# Autodesk Inventor assembly: ModulWalkaNapinajacego
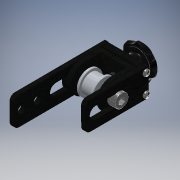
[picture p0: Inventor's stored thumbnail of the model, 180x180]
Saved by Autodesk Inventor 2019 (Build 230136000, 136)
## iProperties
Created: 2020-08-21
Part Number: ModulWalkaNapinajacego
Document SubType Name: Assembly
Designer: estee
Author: estee
## Documents named in this file (9)
- C:\Users\estee\OneDrive\Pulpit\estere\1\MUM\nowygit\Mechanika\Moduł obrotu RET Estera\projejt\projejt\ModulWalkaNapinajacego.iam
- C:\Users\estee\OneDrive\Pulpit\estere\1\MUM\nowygit\Mechanika\Moduł obrotu RET Estera\projejt\projejt\Ramka1.ipt
- C:\Users\estee\OneDrive\Pulpit\estere\1\MUM\nowygit\Mechanika\Moduł obrotu RET Estera\projejt\projejt\Ramka2.ipt
- C:\Users\estee\OneDrive\Pulpit\estere\1\MUM\nowygit\Mechanika\Moduł obrotu RET Estera\projejt\projejt\Ramka3.ipt
- C:\Users\estee\OneDrive\Pulpit\estere\1\MUM\nowygit\Mechanika\Moduł obrotu RET Estera\projejt\projejt\Ramka4.ipt
- C:\Users\estee\OneDrive\Dokumenty\Inventor\Content Center Files\R2019\en-US\BS EN ISO 7045 H\EN ISO 7045 - M2 x 6 - 4.8 - H(1).ipt
- C:\Users\estee\OneDrive\Pulpit\estere\1\MUM\nowygit\Mechanika\Moduł obrotu RET Estera\projejt\projejt\ModulKolaNapinajacego.iam
- C:\Users\estee\OneDrive\Dokumenty\Inventor\Star Knob M6 Male.ipt
- C:\Users\estee\OneDrive\Pulpit\estere\1\MUM\nowygit\Mechanika\Moduł obrotu RET Estera\projejt\projejt\WkretDoNapinacza.ipt
## Components (11 placed, 8 different names)
1. Ramka1:1 — Mate:1, Mate:2, Flush:1, Mate:3, Mate:4, Flush:2, Mate:6, Mate:19, Mate:20, Mate:21, Mate:22
2. Ramka2:1 — Mate:1, Mate:2, Flush:1, Mate:5, Mate:7, Mate:8, Mate:13, Mate:14
3. Ramka3:1 — Mate:3, Mate:4, Flush:2, Mate:9, Mate:10, Mate:11, Mate:12
4. Ramka4:1 — Mate:5, Mate:6, Mate:15, Mate:16
5. BS EN ISO 7045 H - Metric M2 x 6 - 4.8 - H:1 — Mate:7, Mate:13
6. BS EN ISO 7045 H - Metric M2 x 6 - 4.8 - H:2 — Mate:8, Mate:14
7. BS EN ISO 7045 H - Metric M2 x 6 - 4.8 - H:3 — Mate:9, Mate:11
8. BS EN ISO 7045 H - Metric M2 x 6 - 4.8 - H:4 — Mate:10, Mate:12
9. ModulKolaNapinajacego:1 [sub-assembly] — Mate:19, Mate:20
10. Star Knob M6 Male:1 — Mate:15, Mate:16
11. WkretDoNapinacza:1 — Mate:21, Mate:22
## Relationships (22: Mate 20, Flush 2)
- Mate:1: Ramka1:1 ↔ Ramka2:1
- Mate:2: Ramka1:1 ↔ Ramka2:1
- Flush:1: Ramka1:1 ↔ Ramka2:1
- Mate:3: Ramka1:1 ↔ Ramka3:1
- Mate:4: Ramka1:1 ↔ Ramka3:1
- Flush:2: Ramka1:1 ↔ Ramka3:1
- Mate:5: Ramka2:1 ↔ Ramka4:1
- Mate:6: Ramka1:1 ↔ Ramka4:1
- Mate:7: Ramka2:1 ↔ BS EN ISO 7045 H - Metric M2 x 6 - 4.8 - H:1
- Mate:8: Ramka2:1 ↔ BS EN ISO 7045 H - Metric M2 x 6 - 4.8 - H:2
- Mate:9: Ramka3:1 ↔ BS EN ISO 7045 H - Metric M2 x 6 - 4.8 - H:3
- Mate:10: Ramka3:1 ↔ BS EN ISO 7045 H - Metric M2 x 6 - 4.8 - H:4
- Mate:11: Ramka3:1 ↔ BS EN ISO 7045 H - Metric M2 x 6 - 4.8 - H:3
- Mate:12: Ramka3:1 ↔ BS EN ISO 7045 H - Metric M2 x 6 - 4.8 - H:4
- Mate:13: Ramka2:1 ↔ BS EN ISO 7045 H - Metric M2 x 6 - 4.8 - H:1
- Mate:14: Ramka2:1 ↔ BS EN ISO 7045 H - Metric M2 x 6 - 4.8 - H:2
- Mate:15: Ramka4:1 ↔ Star Knob M6 Male:1
- Mate:16: Ramka4:1 ↔ Star Knob M6 Male:1
- Mate:19 (3 mm): Ramka1:1 ↔ ModulKolaNapinajacego:1
- Mate:20: Ramka1:1 ↔ ModulKolaNapinajacego:1
- Mate:21: Ramka1:1 ↔ WkretDoNapinacza:1
- Mate:22: Ramka1:1 ↔ WkretDoNapinacza:1
